# Autodesk Inventor assembly: Assembly8
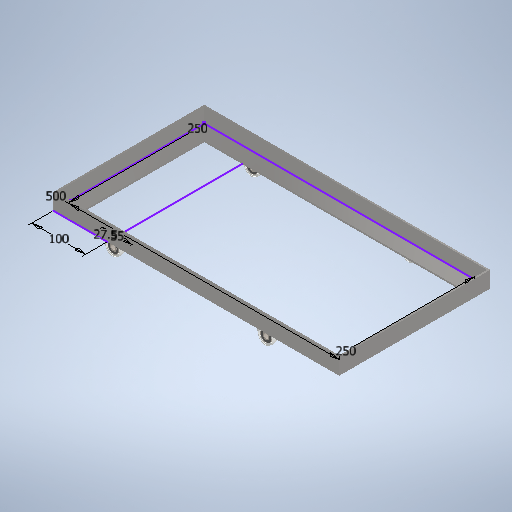
[picture p0: Inventor's stored thumbnail of the model, 512x512]
Saved by Autodesk Inventor 2026.1 (Build 301233020, 233B)
## iProperties
_SolveAssemblyDoc: Frame Generator Solve Assembly
_Version: 25.0.0
Created: 2026-01-19
Part Number: Assembly8
Document SubType Name: Assembly
Designer: user
Author: user
## Documents named in this file (4)
- D:\asu\machine element design\project\design\Assembly8.iam
- D:\asu\machine element design\project\design\Part23.ipt
- D:\asu\machine element design\project\design\Assembly8\Frame\Frame 1768841823111.iam
- C:\Users\user\Downloads\pillow-block-bearing-p08-1.snapshot.17\Pillow Block P08\Pillow Block P08\Pillow Block P08.ipt
## Components (6 placed, 3 different names)
1. Part23:1
2. Frame 1768841823111:1 [sub-assembly] — Mate:1, Mate:2, Mate:3, Mate:4
3. Pillow Block P08:1 — Mate:3
4. Pillow Block P08:2 — Mate:2
5. Pillow Block P08:3 — Mate:4
6. Pillow Block P08:4 — Mate:1
## Relationships (4: Mate 4)
- Mate:1: Frame 1768841823111:1 ↔ Pillow Block P08:4
- Mate:2: Frame 1768841823111:1 ↔ Pillow Block P08:2
- Mate:3: Frame 1768841823111:1 ↔ Pillow Block P08:1
- Mate:4: Frame 1768841823111:1 ↔ Pillow Block P08:3
